# Autodesk Inventor assembly: Assembly1
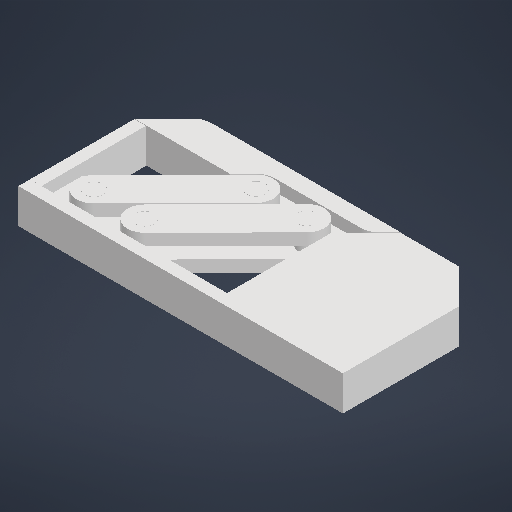
[picture p0: Inventor's stored thumbnail of the model, 512x512]
Saved by Autodesk Inventor 2026.2 (Build 302298000, 298)
## iProperties
Created: 2026-03-23
Part Number: Assembly1
Document SubType Name: Assembly
Designer: Cobble
Author: Cobble
## Documents named in this file (4)
- D:\Archive\Kreative Projekte\Obsidian\Online\Projects\Shot-Dispenser\Design V3\Part 2\Assembly1.iam
- D:\Archive\Kreative Projekte\Obsidian\Online\Projects\Shot-Dispenser\Design V3\Part 2\Basseipt.ipt
- D:\Archive\Kreative Projekte\Obsidian\Online\Projects\Shot-Dispenser\Design V3\Part 2\Connector.ipt
- D:\Archive\Kreative Projekte\Obsidian\Online\Projects\Shot-Dispenser\Design V3\Part 2\Dispenser.ipt
## Components (6 placed, 3 different names)
1. Basseipt:1 — Insert:2, Insert:4, Insert:7, Insert:8
2. Connector:1 — Insert:5, Insert:7
3. Dispenser:1 — Insert:1, Insert:3, Insert:5, Insert:6
4. Connector:2 — Insert:6, Insert:8
5. Connector:3 — Insert:3, Insert:4
6. Connector:4 — Insert:1, Insert:2
## Relationships (8: Insert 8)
- Insert:1: Dispenser:1 ↔ Connector:4
- Insert:2: Basseipt:1 ↔ Connector:4
- Insert:3: Dispenser:1 ↔ Connector:3
- Insert:4: Basseipt:1 ↔ Connector:3
- Insert:5: Connector:1 ↔ Dispenser:1
- Insert:6: Dispenser:1 ↔ Connector:2
- Insert:7: Basseipt:1 ↔ Connector:1
- Insert:8: Basseipt:1 ↔ Connector:2
